# Autodesk Inventor assembly: ロボベース2
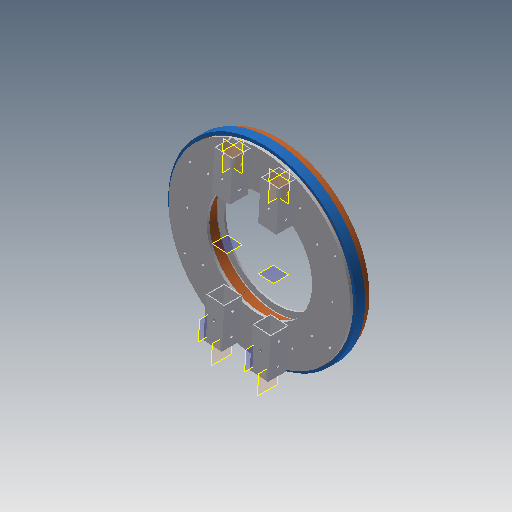
[picture p0: Inventor's stored thumbnail of the model, 512x512]
Saved by Autodesk Inventor 2019.4 (Build 234330000, 330)
## iProperties
Created: 2018-08-09
Part Number: ロボベース2
Document SubType Name: Assembly
Designer: Owner
Mass: 427.035 g
Surface Area: 2119.92 cm^2
Volume: 427.035 cm^3
Density: 1 g/cm^3
Author: Owner
## Documents named in this file (7)
- E:\ロボ研\キャチロボ\キャチロボ2019\アーム2019\2019HDarm\ロボベース2.iam
- E:\ロボ研\キャチロボ\キャチロボ2019\アーム2019\2019HDarm\アームベース円盤.ipt
- E:\ロボ研\キャチロボ\キャチロボ2019\アーム2019\2019HDarm\ベースギア肉.ipt
- E:\ロボ研\キャチロボ\キャチロボ2019\アーム2019\2019HDarm\ベースフレキラックギア.ipt
- E:\ロボ研\キャチロボ\キャチロボ2019\アーム2019\2019HDarm\ロボベース□15.ipt
- E:\ロボ研\キャチロボ\キャチロボ2019\アーム2019\2019HDarm\ベアリングサンド下板.ipt
- E:\ロボ研\キャチロボ\キャチロボ2019\アーム2019\2019HDarm\ベアリングサンド下板alt.ipt
## Components (7 placed, 6 different names)
1. アームベース円盤:1 — 挿入:1, 挿入:2, 挿入:3, 挿入:4
2. ベースギア肉:1
3. ベースフレキラックギア:1
4. ロボベース□15:1 — 挿入:3, 挿入:4
5. ロボベース□15:2 — 挿入:1, 挿入:2
6. ベアリングサンド下板:1
7. ベアリングサンド下板alt:1
## Relationships (4: Insert 4)
- 挿入:1 [Insert]: アームベース円盤:1 ↔ ロボベース□15:2
- 挿入:2 [Insert]: アームベース円盤:1 ↔ ロボベース□15:2
- 挿入:3 [Insert]: アームベース円盤:1 ↔ ロボベース□15:1
- 挿入:4 [Insert]: アームベース円盤:1 ↔ ロボベース□15:1
